# Autodesk Inventor assembly: 000.100 - Манипулятор
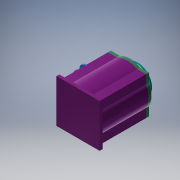
[picture p0: Inventor's stored thumbnail of the model, 180x180]
Saved by Autodesk Inventor 2019 (Build 230136000, 136)
## iProperties
Created: 2020-03-17
Part Number: 000.100 - Манипулятор
Material: Типовые
Document SubType Name: Assembly
Designer: Петров Иван
Author: Петров Иван
## Documents named in this file (5)
- E:\IVAN\Ivan_desktop\Kvantorium\Competitions\INOP_2020\hardware\SCARA(Dynamixels)\000.100 - Манипулятор.iam
- E:\IVAN\Ivan_desktop\Kvantorium\Competitions\INOP_2020\hardware\SCARA(Dynamixels)\000.200 - Основание.iam
- E:\IVAN\Ivan_desktop\Kvantorium\Competitions\INOP_2020\hardware\SCARA(Dynamixels)\000.300 - Рычаг 1.iam
- E:\IVAN\Ivan_desktop\Kvantorium\Competitions\INOP_2020\hardware\SCARA(Dynamixels)\000.400 - Рычаг 2.iam
- E:\IVAN\Ivan_desktop\Kvantorium\Competitions\INOP_2020\hardware\SCARA(Dynamixels)\000.400 - Рычаг 2\000.500 - Подъемная платформа.iam
## Components (4 placed, 4 different names)
1. 000.200 - Основание:1 [sub-assembly] — Совмещение:1, Совмещение:2, Совмещение:3, Угол:1
2. 000.300 - Рычаг 1:1 [sub-assembly] — Совмещение:1, Совмещение:2, Совмещение:3, Совмещение:4, Совмещение:5, Совмещение:6, Угол:1, Угол:2
3. 000.400 - Рычаг 2:1 [sub-assembly] — Совмещение:4, Совмещение:5, Совмещение:6, Угол:2, Совмещение:8, Совмещение:9
4. 000.500 - Подъемная платформа:1 [sub-assembly] — Совмещение:8, Совмещение:9
## Relationships (10: Mate 8, Angle 2)
- Совмещение:1 [Mate]: 000.200 - Основание:1 ↔ 000.300 - Рычаг 1:1
- Совмещение:2 [Mate]: 000.200 - Основание:1 ↔ 000.300 - Рычаг 1:1
- Совмещение:3 [Mate]: 000.200 - Основание:1 ↔ 000.300 - Рычаг 1:1
- Совмещение:4 [Mate]: 000.300 - Рычаг 1:1 ↔ 000.400 - Рычаг 2:1
- Совмещение:5 [Mate]: 000.300 - Рычаг 1:1 ↔ 000.400 - Рычаг 2:1
- Совмещение:6 [Mate]: 000.300 - Рычаг 1:1 ↔ 000.400 - Рычаг 2:1
- Угол:1 [Angle] (296.57 deg): 000.200 - Основание:1 ↔ 000.300 - Рычаг 1:1
- Угол:2 [Angle] (0 deg): 000.300 - Рычаг 1:1 ↔ 000.400 - Рычаг 2:1
- Совмещение:8 [Mate]: 000.400 - Рычаг 2:1 ↔ 000.500 - Подъемная платформа:1
- Совмещение:9 [Mate]: 000.400 - Рычаг 2:1 ↔ 000.500 - Подъемная платформа:1
